# Autodesk Inventor assembly: Asamblare
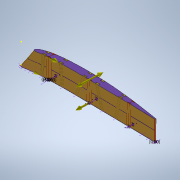
[picture p0: Inventor's stored thumbnail of the model, 180x180]
Saved by Autodesk Inventor 2022 (Build 260153000, 153)
## iProperties
Created: 2022-05-27
Part Number: Asamblare
Document SubType Name: Assembly
Designer: 40742
Title: Perfection
Author: 40742
## Documents named in this file (10)
- C:\Users\40742\Documents\Inventor\TASD\Asamblare.iam
- C:\Users\40742\Documents\Inventor\TASD\lonjeron.ipt
- C:\Users\40742\Documents\Inventor\TASD\Nervuri.ipt
- C:\Users\40742\Documents\Inventor\TASD\Lise (2).ipt
- C:\Users\40742\Documents\Inventor\TASD\Invelis.ipt
- C:\Users\40742\Documents\Inventor\TASD\Asamblare\AIP\FEA\dzf3gcv8g.fins
- C:\Users\40742\Documents\Inventor\TASD\Asamblare\AIP\FEA\dzf3gcv8g.fsat
- C:\Users\40742\Documents\Inventor\TASD\Asamblare\AIP\FEA\dzf3gcv8g.ftes
- C:\Users\40742\Documents\Inventor\TASD\Asamblare\AIP\FEA\dzf3gcv8g.fwiz
- C:\Users\40742\Documents\Inventor\TASD\Asamblare\AIP\FEA\dzf3gcvcw.fmsh
## Components (4 placed, 1 different names)
1. Profil:1 — Mate:1, Flush:1, Flush:2, Rigid:1
2. Profil:2 — Mate:1, Flush:1, Flush:2, Flush:3, Flush:4
3. Profil:3 — Flush:3
4. Profil:4 — Flush:4, Rigid:1
## Relationships (6: Flush 4, Mate 1, WeldJoint 1)
- Mate:1: Profil:1 ↔ Profil:2
- Flush:1: Profil:1 ↔ Profil:2
- Flush:2: Profil:1 ↔ Profil:2
- Flush:3: Profil:2 ↔ Profil:3
- Flush:4: Profil:2 ↔ Profil:4
- Rigid:1 [WeldJoint]: Profil:1 ↔ Profil:4
## Named parameters: sa_0 = 39990.2, sa_1 = 2.99949e+06, sa_2 = -38552.2, sa_3 = 40858.3, sa_4 = 2.99947e+06, sa_5 = -38557.6, sa_6 = -340.941, sa_7 = -24996, sa_8 = 287.956, sa_9 = -333.35, sa_10 = -24996.1, sa_11 = 287.906, sa_12 = 7942.89, sa_13 = 39.0914, sa_14 = -953.367, sa_15 = 7959.98, sa_16 = 60.7893, sa_17 = 796.842
note: some values were not read from the file. Shown as the stored number, unit unknown: "sa_0", "sa_1", "sa_2", "sa_3", "sa_4", "sa_5", "sa_6", "sa_7", "sa_8", "sa_9", "sa_10", "sa_11", "sa_12", "sa_13", "sa_14", "sa_15", "sa_16", "sa_17".
